# Autodesk Inventor assembly: heater_case
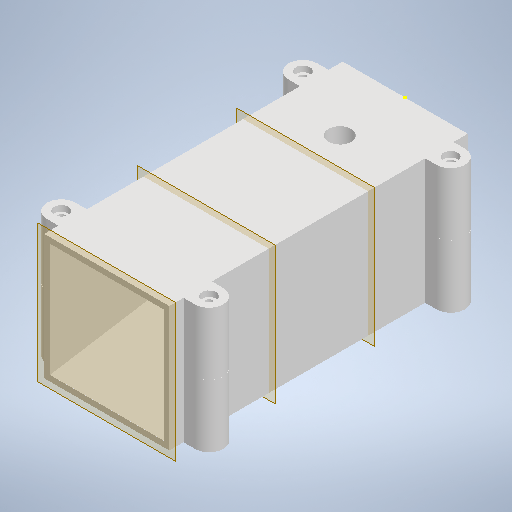
[picture p0: Inventor's stored thumbnail of the model, 512x512]
Saved by Autodesk Inventor 2025.4 (Build 294407000, 407)
## iProperties
Created: 2025-12-17
Part Number: heater_case
Document SubType Name: Assembly
Designer: FOX
Author: FOX
## Documents named in this file (3)
- C:\Users\FOX\Documents\GIT\Szklarnia_PBL-Krol-2025-26\Inventor\heater_case.iam
- C:\Users\FOX\Documents\GIT\Szklarnia_PBL-Krol-2025-26\Inventor\heater_case_bottom.ipt
- C:\Users\FOX\Documents\GIT\Szklarnia_PBL-Krol-2025-26\Inventor\heater_case_top.ipt
## Components (2 placed, 2 different names)
1. heater_case_bottom:1 — Zestawiające:1, Równoległe:1, Równoległe:2
2. heater_case_top:1 — Zestawiające:1, Równoległe:1, Równoległe:2
## Relationships (3: Flush 2, Mate 1)
- Zestawiające:1 [Mate]: heater_case_bottom:1 ↔ heater_case_top:1
- Równoległe:1 [Flush]: heater_case_bottom:1 ↔ heater_case_top:1
- Równoległe:2 [Flush]: heater_case_bottom:1 ↔ heater_case_top:1
